# Autodesk Inventor assembly: bellows_latest
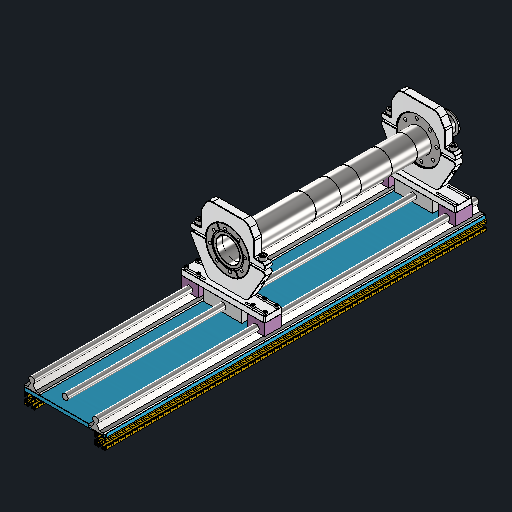
[picture p0: Inventor's stored thumbnail of the model, 512x512]
Saved by Autodesk Inventor 2027.1 (Build 311270010, 270A)
## iProperties
Created: 2026-06-04
Part Number: bellows_latest
Document SubType Name: Assembly
Designer: shusu
Author: shusu
## Documents named in this file (17)
- C:\Users\queezz\Dropbox\Drawings\pihti-cad\bwllows-probe\sliding-assembly.iam
- C:\Users\queezz\Dropbox\Drawings\pihti-cad\bwllows-probe\rail bwllows probe.ipt
- C:\Users\queezz\Dropbox\Drawings\pihti-cad\bwllows-probe\flange-camp-114.ipt
- C:\Users\queezz\Dropbox\Drawings\pihti-cad\bwllows-probe\bellows_flange.ipt
- C:\Users\queezz\Dropbox\Drawings\pihti-cad\bwllows-probe\linearbearing.ipt
- C:\Users\queezz\Dropbox\Drawings\pihti-cad\bwllows-probe\instead-of-bellows.ipt
- C:\Users\queezz\Dropbox\Drawings\pihti-cad\bwllows-probe\clamp-foot.ipt
- C:\Users\queezz\Dropbox\Drawings\pihti-cad\bwllows-probe\Al-profile-30x30-L1000.ipt
- C:\Users\queezz\Dropbox\Drawings\pihti-cad\ContentCenter\Aluminium-profiles\Al-profile-30x30.ipt
- C:\Users\queezz\Dropbox\Drawings\pihti-cad\bwllows-probe\base-plate-for-bellows.ipt
- C:\Users\queezz\Dropbox\Drawings\pihti-cad\ContentCenter\Fastners\M6x16-SHCS.ipt
- C:\Users\queezz\Dropbox\Drawings\pihti-cad\ContentCenter\Fastners\M5x20-SHCS.ipt
- C:\Users\queezz\Dropbox\Drawings\pihti-cad\ContentCenter\CF-KF-adapters\ICF70_to_KF40.ipt
- C:\Users\queezz\Dropbox\Drawings\pihti-cad\bwllows-probe\CF114-CF70-zero-length-adappter.ipt
- C:\Users\queezz\Documents\Inventor\Content Center Files\R2027\en-US\AS 1420\AS 1420 - 1973 - M10 x 30.ipt
- C:\Users\queezz\Dropbox\Drawings\pihti-cad\bwllows-probe\M16-lead-screw.ipt
- C:\Users\queezz\Dropbox\Drawings\pihti-cad\bwllows-probe\lead-screw-nut-preview.ipt
## Components (40 placed, 15 different names)
1. rail:1 — Mate:1, Mate:4, Mate:9
2. rail:2 — Mate:2, Mate:3, Mate:9, Mate:16, Flush:12, Flush:20
3. flange-camp-114:1 — Flush:8, Mate:12, Mate:14, Rigid:15, Rigid:19, Rigid:20
4. flange-camp-114:2 — Mate:24, Mate:25, Flush:17, Rigid:16, Rigid:17, Rigid:18
5. bellows_flange:1 — Rigid:4, Mate:15, Rigid:16
6. bellows_flange:2 — Rigid:3, Mate:15, Rigid:14, Rigid:15
7. linearbearing:1 — Mate:4, Flush:2, Flush:18, Rotational:1, Rotational:2, Rotational:3, Rotational:4
8. linearbearing:2 — Mate:2, Flush:1, Flush:3
9. linearbearing:3 — Mate:3, Flush:2, Mate:8, Flush:19, Rigid:9, Rotational:5, Rigid:10, Rigid:11
10. linearbearing:4 — Mate:1, Flush:1, Flush:3, Flush:9, Flush:10
11. instead-of-bellows:1 — Rigid:3, Mate:5, Mate:10, Mate:19, Mate:22
12. instead-of-bellows:2 — Rigid:4, Mate:5, Mate:20, Mate:21
13. clamp-foot:1 — Mate:8, Rigid:5, Rigid:6, Mate:24, Mate:25, Flush:17, Flush:18, Flush:19, Rigid:21
14. clamp-foot:2 — Flush:8, Mate:12, Flush:9, Clamp foot 2 bottom seated on assembly XY, Flush:10, Mate:14, Rigid:7, Rigid:8, Rigid:22
15. Al-profile-30x30-L1000:1 — Mate:18, Flush:13, Flush:16
16. Al-profile-30x30-L1000:2 — Mate:17, Flush:14, Flush:15
17. base-plate-for-bellows:1 — Mate:16, Flush:11, Flush:12, Mate:17, Mate:18, Flush:13, Flush:14, Flush:15, Flush:16
18. instead-of-bellows:3 — Mate:20, Mate:21, Mate:23
19. instead-of-bellows:4 — Mate:19, Mate:22, Mate:23
20. ICF70_to_KF40:1 — Rotational:6
21. CF114-CF70-zero-length-adappter:1 — Rigid:14, Rotational:6
22. M16-lead-screw:1 — Mate:26, Flush:20
23. lead-screw-nut-preview:1 — Mate:26, Rigid:21
24. lead-screw-nut-preview:2 — Rigid:22
25. AS 1420 - Metric M10 x 30:1 — Rigid:19
26. AS 1420 - Metric M10 x 30:2 — Rigid:20
27. AS 1420 - Metric M10 x 30:3 — Rigid:17
28. AS 1420 - Metric M10 x 30:4 — Rigid:18
29. JIS B 1176 - Metric M6 x 16:2 — Rigid:6
30. JIS B 1176 - Metric M6 x 16:3 — Rigid:7
31. JIS B 1176 - Metric M6 x 16:4 — Rigid:8
32. AS 1420 - Metric M5 x 20:1 — Rotational:1
33. AS 1420 - Metric M5 x 20:2 — Rotational:3
34. AS 1420 - Metric M5 x 20:3 — Rotational:2
35. AS 1420 - Metric M5 x 20:4 — Rigid:11
36. AS 1420 - Metric M5 x 20:5 — Rigid:10
37. AS 1420 - Metric M5 x 20:6 — Rotational:5
38. AS 1420 - Metric M5 x 20:7 — Rotational:4
39. AS 1420 - Metric M5 x 20:8 — Rigid:9
40. JIS B 1176 - Metric M6 x 16:1 — Rigid:5
## Relationships (63: Mate 23, WeldJoint 18, Flush 16, RevoluteJoint 6)
- Mate:1: rail:1 ↔ linearbearing:4
- Mate:2: rail:2 ↔ linearbearing:2
- Mate:3: rail:2 ↔ linearbearing:3
- Mate:4: rail:1 ↔ linearbearing:1
- Flush:1: linearbearing:2 ↔ linearbearing:4
- Flush:2: linearbearing:1 ↔ linearbearing:3
- Flush:3: linearbearing:2 ↔ linearbearing:4
- Rigid:3 [WeldJoint]: bellows_flange:2 ↔ instead-of-bellows:1
- Rigid:4 [WeldJoint]: bellows_flange:1 ↔ instead-of-bellows:2
- Mate:5: instead-of-bellows:1 ↔ instead-of-bellows:2
- Mate:8: linearbearing:3 ↔ clamp-foot:1
- Mate:9 (175 mm): rail:1 ↔ rail:2
- Mate:10: instead-of-bellows:1
- Flush:8: flange-camp-114:1 ↔ clamp-foot:2
- Mate:12: flange-camp-114:1 ↔ clamp-foot:2
- Flush:9: linearbearing:4 ↔ clamp-foot:2
- Clamp foot 2 bottom seated on assembly XY [Mate]: clamp-foot:2
- Flush:10: linearbearing:4 ↔ clamp-foot:2
- Mate:14: flange-camp-114:1 ↔ clamp-foot:2
- Mate:15 (-650 mm): bellows_flange:1 ↔ bellows_flange:2
- Mate:16: rail:2 ↔ base-plate-for-bellows:1
- Flush:11: base-plate-for-bellows:1
- Flush:12: rail:2 ↔ base-plate-for-bellows:1
- Mate:17: Al-profile-30x30-L1000:2 ↔ base-plate-for-bellows:1
- Mate:18: Al-profile-30x30-L1000:1 ↔ base-plate-for-bellows:1
- Flush:13: Al-profile-30x30-L1000:1 ↔ base-plate-for-bellows:1
- Flush:14: Al-profile-30x30-L1000:2 ↔ base-plate-for-bellows:1
- Flush:15: Al-profile-30x30-L1000:2 ↔ base-plate-for-bellows:1
- Flush:16: Al-profile-30x30-L1000:1 ↔ base-plate-for-bellows:1
- Mate:19: instead-of-bellows:1 ↔ instead-of-bellows:4
- Mate:20: instead-of-bellows:2 ↔ instead-of-bellows:3
- Mate:21: instead-of-bellows:2 ↔ instead-of-bellows:3
- Mate:22 (-200 mm): instead-of-bellows:1 ↔ instead-of-bellows:4
- Mate:23: instead-of-bellows:3 ↔ instead-of-bellows:4
- Rigid:5 [WeldJoint]: clamp-foot:1 ↔ JIS B 1176 - Metric M6 x 16:1
- Rigid:6 [WeldJoint]: clamp-foot:1 ↔ JIS B 1176 - Metric M6 x 16:2
- Rigid:7 [WeldJoint]: clamp-foot:2 ↔ JIS B 1176 - Metric M6 x 16:3
- Rigid:8 [WeldJoint]: clamp-foot:2 ↔ JIS B 1176 - Metric M6 x 16:4
- Mate:24: flange-camp-114:2 ↔ clamp-foot:1
- Mate:25: flange-camp-114:2 ↔ clamp-foot:1
- Flush:17: flange-camp-114:2 ↔ clamp-foot:1
- Flush:18: linearbearing:1 ↔ clamp-foot:1
- Rotational:1 [RevoluteJoint] (15 mm): linearbearing:1 ↔ AS 1420 - Metric M5 x 20:1
- Rotational:2 [RevoluteJoint] (15 mm): linearbearing:1 ↔ AS 1420 - Metric M5 x 20:3
- Rotational:3 [RevoluteJoint] (15 mm): linearbearing:1 ↔ AS 1420 - Metric M5 x 20:2
- Rotational:4 [RevoluteJoint] (15 mm): linearbearing:1 ↔ AS 1420 - Metric M5 x 20:7
- Flush:19: linearbearing:3 ↔ clamp-foot:1
- Rigid:9 [WeldJoint] (15 mm): linearbearing:3 ↔ AS 1420 - Metric M5 x 20:8
- Rotational:5 [RevoluteJoint] (15 mm): linearbearing:3 ↔ AS 1420 - Metric M5 x 20:6
- Rigid:10 [WeldJoint] (15 mm): linearbearing:3 ↔ AS 1420 - Metric M5 x 20:5
- Rigid:11 [WeldJoint] (15 mm): linearbearing:3 ↔ AS 1420 - Metric M5 x 20:4
- Rigid:14 [WeldJoint]: bellows_flange:2 ↔ CF114-CF70-zero-length-adappter:1
- Rotational:6 [RevoluteJoint]: ICF70_to_KF40:1 ↔ CF114-CF70-zero-length-adappter:1
- Rigid:15 [WeldJoint]: flange-camp-114:1 ↔ bellows_flange:2
- Rigid:16 [WeldJoint]: flange-camp-114:2 ↔ bellows_flange:1
- Rigid:17 [WeldJoint]: flange-camp-114:2 ↔ AS 1420 - Metric M10 x 30:3
- Rigid:18 [WeldJoint]: flange-camp-114:2 ↔ AS 1420 - Metric M10 x 30:4
- Rigid:19 [WeldJoint]: flange-camp-114:1 ↔ AS 1420 - Metric M10 x 30:1
- Rigid:20 [WeldJoint]: flange-camp-114:1 ↔ AS 1420 - Metric M10 x 30:2
- Mate:26: M16-lead-screw:1 ↔ lead-screw-nut-preview:1
- Flush:20: rail:2 ↔ M16-lead-screw:1
- Rigid:21 [WeldJoint]: clamp-foot:1 ↔ lead-screw-nut-preview:1
- Rigid:22 [WeldJoint]: clamp-foot:2 ↔ lead-screw-nut-preview:2
